# Autodesk Inventor assembly: EVK4 – HD
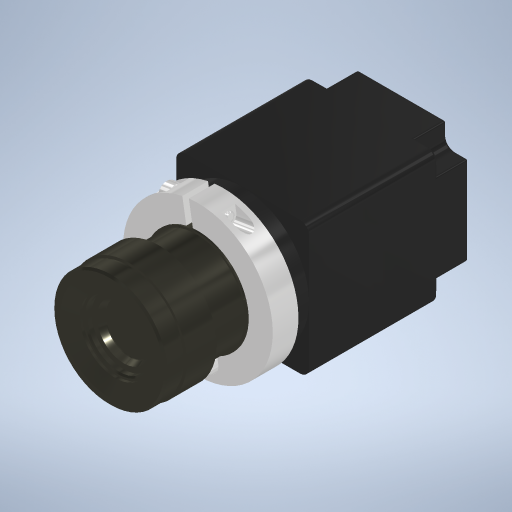
[picture p0: Inventor's stored thumbnail of the model, 512x512]
Saved by Autodesk Inventor 2023 (Build 270158000, 158)
## iProperties
Created: 2022-12-16
Part Number: EVK4 – HD
Document SubType Name: Assembly
Designer: ASARe-DAQ-PC
Sending System: SolidWorks 2019
Last Author: ASARe-DAQ-PC
Last Saved: 2022-12-16
Author: ASARe-DAQ-PC
## Documents named in this file (4)
- D:\EB camera\model of EB camera\for manufacture\EVK4 – HD.iam
- D:\EB camera\model of EB camera\for manufacture\EVK4 – HD.ipt
- D:\EB camera\model of EB camera\for manufacture\User Library-USB - C.ipt
- D:\EB camera\model of EB camera\for manufacture\Camera Lens.iam
## Components (3 placed, 3 different names)
1. EVK4 – HD:1 — Insert:1
2. User Library-USB - C:1
3. Camera Lens:1 [sub-assembly] — Insert:1
## Relationships (1: Insert 1)
- Insert:1: EVK4 – HD:1 ↔ Camera Lens:1
